# Autodesk Inventor assembly: Bearing Block
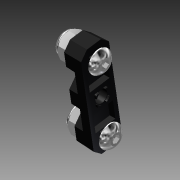
[picture p0: Inventor's stored thumbnail of the model, 180x180]
Saved by Autodesk Inventor 2012 (Build 160160000, 160)
## iProperties
Created: 2011-04-17
Part Number: Bearing Block
Document SubType Name: Assembly
Designer: Andrew
Mass: 5.39498 g
Surface Area: 21.8098 cm^2
Volume: 1.98215 cm^3
Density: 2.72178 g/cm^3
Author: Andrew
## Documents named in this file (3)
- C:\Users\Wade\Documents\1103 Robot - CAD Assembly\Bearing Block.iam
- C:\Users\Wade\Documents\1103 Robot - CAD Assembly\Flat Bearing Block.ipt
- C:\Users\Wade\Documents\1103 Robot - CAD Assembly\2x .5'' Screw & Nylock Nut.iam
## Components (2 placed, 2 different names)
1. Flat Bearing Block:1 — Mate:1, Mate:2, Mate:3
2. 2x .5'' Screw & Nylock Nut:1 [sub-assembly] — Mate:1, Mate:2, Mate:3
## Relationships (3: Mate 3)
- Mate:1: Flat Bearing Block:1 ↔ 2x .5'' Screw & Nylock Nut:1
- Mate:2: Flat Bearing Block:1 ↔ 2x .5'' Screw & Nylock Nut:1
- Mate:3: Flat Bearing Block:1 ↔ 2x .5'' Screw & Nylock Nut:1
